# Autodesk Inventor assembly: Harmonic Drive - My Assembly
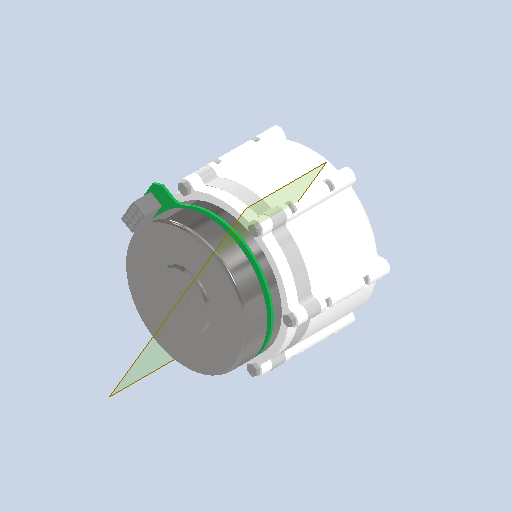
[picture p0: Inventor's stored thumbnail of the model, 512x512]
Saved by Autodesk Inventor 2023.2 (Build 272271000, 271)
## iProperties
Created: 2023-01-17
Part Number: Harmonic Drive - My Assembly
Document SubType Name: Assembly
Designer: Letícia
Author: Letícia
## Documents named in this file (27)
- C:\Users\User\Desktop\IC - Prof. Rafael\CADs\Redução Harmônica\HowToMechatronics\Harmonic Drive - PROJETO\Harmonic Drive - My Assembly.iam
- C:\Users\User\Desktop\IC - Prof. Rafael\CADs\Redução Harmônica\HowToMechatronics\Harmonic Drive - PROJETO\Housing.ipt
- C:\Users\User\Desktop\IC - Prof. Rafael\CADs\Redução Harmônica\HowToMechatronics\Harmonic Drive - PROJETO\4668K269.ipt
- C:\Users\User\Desktop\IC - Prof. Rafael\CADs\Redução Harmônica\HowToMechatronics\Harmonic Drive - PROJETO\BearingSpacer.ipt
- C:\Users\User\Desktop\IC - Prof. Rafael\CADs\Redução Harmônica\HowToMechatronics\Harmonic Drive - PROJETO\BearingSpacer2.ipt
- C:\Users\User\Desktop\IC - Prof. Rafael\CADs\Redução Harmônica\HowToMechatronics\Harmonic Drive - PROJETO\Spline output.ipt
- C:\Users\User\Desktop\IC - Prof. Rafael\CADs\Redução Harmônica\HowToMechatronics\Harmonic Drive - PROJETO\92010A230.ipt
- C:\Users\User\Desktop\IC - Prof. Rafael\CADs\Redução Harmônica\HowToMechatronics\Harmonic Drive - PROJETO\93475A230.ipt
- C:\Users\User\Desktop\IC - Prof. Rafael\CADs\Redução Harmônica\HowToMechatronics\Harmonic Drive - PROJETO\90576A103.ipt
- C:\Users\User\Desktop\IC - Prof. Rafael\CADs\Redução Harmônica\HowToMechatronics\Harmonic Drive - PROJETO\Output shaft.ipt
- C:\Users\User\Desktop\IC - Prof. Rafael\CADs\Redução Harmônica\HowToMechatronics\Harmonic Drive - PROJETO\91415A020.ipt
- C:\Users\User\Desktop\IC - Prof. Rafael\CADs\Redução Harmônica\HowToMechatronics\Harmonic Drive - PROJETO\92010A242.ipt
- C:\Users\User\Desktop\IC - Prof. Rafael\CADs\Redução Harmônica\HowToMechatronics\Harmonic Drive - PROJETO\Output.ipt
- C:\Users\User\Desktop\IC - Prof. Rafael\CADs\Redução Harmônica\HowToMechatronics\Harmonic Drive - PROJETO\91280A132.ipt
- C:\Users\User\Desktop\IC - Prof. Rafael\CADs\Redução Harmônica\HowToMechatronics\Harmonic Drive - PROJETO\Flex Spline.ipt
- C:\Users\User\Desktop\IC - Prof. Rafael\CADs\Redução Harmônica\HowToMechatronics\Harmonic Drive - PROJETO\Circular Spline.ipt
- C:\Users\User\Desktop\IC - Prof. Rafael\CADs\Redução Harmônica\HowToMechatronics\Harmonic Drive - PROJETO\Wave Generator p1.ipt
- C:\Users\User\Desktop\IC - Prof. Rafael\CADs\Redução Harmônica\HowToMechatronics\Harmonic Drive - PROJETO\Wave Generator p2.ipt
- C:\Users\User\Desktop\IC - Prof. Rafael\CADs\Redução Harmônica\HowToMechatronics\Harmonic Drive - PROJETO\4668K117.ipt
- C:\Users\User\Desktop\IC - Prof. Rafael\CADs\Redução Harmônica\HowToMechatronics\Harmonic Drive - PROJETO\92010A126.ipt
- C:\Users\User\Desktop\IC - Prof. Rafael\CADs\Redução Harmônica\HowToMechatronics\Harmonic Drive - PROJETO\90576A102.ipt
- C:\Users\User\Desktop\IC - Prof. Rafael\CADs\Redução Harmônica\HowToMechatronics\Harmonic Drive - PROJETO\Motor mount - Lid.ipt
- C:\Users\User\Desktop\IC - Prof. Rafael\CADs\Redução Harmônica\HowToMechatronics\Harmonic Drive - PROJETO\93695A120.ipt
- C:\Users\User\Desktop\IC - Prof. Rafael\CADs\Redução Harmônica\HowToMechatronics\Harmonic Drive - PROJETO\92605A102.ipt
- C:\Users\User\Desktop\IC - Prof. Rafael\Bancada\Motor Maxon323772_EC90fl_90W_A.ipt
- C:\Users\User\Documents\Inventor\Content Center Files\R2023\pt-BR\ANSI B18.6.5M(07)\ANSI B18.6.5M - 4.8x1.6 x 10(14).ipt
- C:\Users\User\Desktop\IC - Prof. Rafael\CADs\Redução Harmônica\HowToMechatronics\Harmonic Drive - PROJETO\91280A148.ipt
## Components (128 placed, 26 different names)
1. Housing:1 — Coincidente:1, Coincidente:2, Coincidente:4, Coincidente:8, Coincidente:11, Coincidente:12, Coincidente:13, Coincidente:14, Coincidente:41, Coincidente:42, Coincidente:43, Coincidente:44, Coincidente:45, Coincidente:143, Coincidente:144
2. 4668K269:1 — Coincidente:1, Coincidente:2, Coincidente:3, Coincidente:5, Coincidente:6, Coincidente:10
3. BearingSpacer:1 — Coincidente:3, Coincidente:4, Coincidente:7
4. BearingSpacer2:1 — Coincidente:5, Coincidente:6
5. Spline output:1 — Coincidente:9, Coincidente:10, Coincidente:18, Coincidente:19, Coincidente:20, Coincidente:21, Coincidente:22, Coincidente:23, Coincidente:32, Coincidente:34, Coincidente:35, Coincidente:36
6. Output shaft:1 — Coincidente:18, Coincidente:19, Coincidente:20, Coincidente:21, Coincidente:22, Coincidente:23, Coincidente:24, Coincidente:25, Coincidente:26, Coincidente:27, Coincidente:28, Coincidente:29
7. Output:1 — Coincidente:27, Coincidente:28, Coincidente:29, Coincidente:30, Coincidente:31
8. Flex Spline:1 — Coincidente:36, Coincidente:37, Coincidente:38, Coincidente:39
9. Circular Spline:1 — Coincidente:41, Coincidente:42, Coincidente:43, Coincidente:136, Coincidente:139, Coincidente:140, Coincidente:141
10. Wave Generator p1:1 — Coincidente:46, Coincidente:47, Coincidente:48, Coincidente:49, Coincidente:50, Coincidente:51, Coincidente:52, Coincidente:53, Coincidente:54, Coincidente:55, Coincidente:56, Coincidente:57, Coincidente:58, Coincidente:59, Coincidente:60, Coincidente:61, Coincidente:62, Coincidente:63, Coincidente:64, Coincidente:65, Coincidente:66, Coincidente:67, Coincidente:68, Coincidente:69, Coincidente:70, Coincidente:71, Coincidente:72, Coincidente:73, Coincidente:74, Coincidente:75, Coincidente:76, Coincidente:77, Coincidente:78, Coincidente:79, Coincidente:80, Coincidente:81, Coincidente:82, Coincidente:83, Coincidente:84, Coincidente:85, Coincidente:86, Coincidente:87, Coincidente:88, Coincidente:109, Coincidente:110, Coincidente:111, Coincidente:112, Coincidente:114, Coincidente:116, Coincidente:117, Coincidente:118, Coincidente:119, Coincidente:120, Coincidente:121, Coincidente:122, Coincidente:134, Coincidente:135
11. Wave Generator p2:1 — Coincidente:66, Coincidente:67, Coincidente:68, Coincidente:90, Coincidente:92, Coincidente:94, Coincidente:96, Coincidente:98, Coincidente:100, Coincidente:102, Coincidente:104, Coincidente:106, Coincidente:108, Coincidente:126, Coincidente:127, Coincidente:138
12. 4668K117:8 — Coincidente:46, Coincidente:47
13. 4668K117:9 — Coincidente:48, Coincidente:49
14. 4668K117:10 — Coincidente:64, Coincidente:65
15. 4668K117:11 — Coincidente:62, Coincidente:63
16. 4668K117:12 — Coincidente:60, Coincidente:61
17. 4668K117:13 — Coincidente:58, Coincidente:59
18. 4668K117:14 — Coincidente:56, Coincidente:57
19. 4668K117:15 — Coincidente:54, Coincidente:55
20. 4668K117:16 — Coincidente:52, Coincidente:53
21. 4668K117:17 — Coincidente:50, Coincidente:51
22. 92010A126:1 — Coincidente:75, Coincidente:76, Coincidente:107
23. 92010A126:2 — Coincidente:73, Coincidente:74, Coincidente:97
24. 92010A126:3 — Coincidente:71, Coincidente:72, Coincidente:95
25. 92010A126:4 — Coincidente:69, Coincidente:70, Coincidente:93
26. 92010A126:5 — Coincidente:87, Coincidente:88, Coincidente:89
27. 92010A126:6 — Coincidente:85, Coincidente:86, Coincidente:91
28. 92010A126:7 — Coincidente:83, Coincidente:84, Coincidente:105
29. 92010A126:8 — Coincidente:81, Coincidente:82, Coincidente:103
30. 92010A126:9 — Coincidente:79, Coincidente:80, Coincidente:101
31. 92010A126:10 — Coincidente:77, Coincidente:78, Coincidente:99
32. 90576A102:1 — Coincidente:89, Coincidente:90
33. 90576A102:2 — Coincidente:91, Coincidente:92
34. 90576A102:3 — Coincidente:105, Coincidente:106
35. 90576A102:4 — Coincidente:103, Coincidente:104
36. 90576A102:5 — Coincidente:101, Coincidente:102
37. 90576A102:6 — Coincidente:99, Coincidente:100
38. 90576A102:7 — Coincidente:107, Coincidente:108
39. 90576A102:8 — Coincidente:97, Coincidente:98
40. 90576A102:9 — Coincidente:95, Coincidente:96
41. 90576A102:10 — Coincidente:93, Coincidente:94
42. Motor mount - Lid:1 — Coincidente:128, Coincidente:129, Coincidente:130, Coincidente:131, Coincidente:132, Coincidente:133, Coincidente:134, Coincidente:136, Coincidente:139, Coincidente:140, Coincidente:142
43. 93695A120:1 — Coincidente:109, Coincidente:110, Coincidente:113
44. 93695A120:2 — Coincidente:111, Coincidente:112, Coincidente:115
45. 92605A102:1 — Coincidente:113, Coincidente:114
46. 92605A102:2 — Coincidente:115, Coincidente:116
47. 92010A126:11 — Coincidente:119, Coincidente:120, Coincidente:123
48. 92010A126:12 — Coincidente:121, Coincidente:122, Coincidente:137
49. 92010A126:13 — Coincidente:117, Coincidente:118, Coincidente:125
50. 90576A102:11 — Coincidente:123, Coincidente:127
51. 90576A102:13 — Coincidente:125, Coincidente:126
52. Motor Maxon323772_EC90fl_90W_A:1 — Coincidente:128, Coincidente:129, Coincidente:130, Coincidente:135, Flush:1
53. Parafuso Phillips para chapa de cabeça escareada reta - Tipo BT - Tipo IA - Métrica 4.8x1.6 x 10:1 — Coincidente:131
54. Parafuso Phillips para chapa de cabeça escareada reta - Tipo BT - Tipo IA - Métrica 4.8x1.6 x 10:2 — Coincidente:132
55. Parafuso Phillips para chapa de cabeça escareada reta - Tipo BT - Tipo IA - Métrica 4.8x1.6 x 10:3 — Coincidente:133
56. 90576A102:14 — Coincidente:137, Coincidente:138
57. 92010A230:1 — Coincidente:11, Coincidente:12, Coincidente:13, Coincidente:15, Coincidente:17
58. 4668K269:2 — Coincidente:7, Coincidente:8, Coincidente:9
59. 92010A230:7
60. 4668K269:3
61. 92010A230:8
62. 4668K269:4
63. 92010A230:9
64. 4668K269:5
65. 92010A230:10
66. 4668K269:6
67. 92010A230:11
68. 4668K269:7
69. 93475A230:1 — Coincidente:14, Coincidente:15, Coincidente:16
70. 93475A230:2
71. 93475A230:3
72. 93475A230:4
73. 93475A230:5
74. 93475A230:6
75. 90576A103:1 — Coincidente:16, Coincidente:17
76. 90576A103:2
77. 90576A103:3
78. 90576A103:4
79. 90576A103:5
80. 90576A103:6
81. 91415A020:1 — Coincidente:24, Coincidente:25, Coincidente:26
82. 91415A020:2
83. 91415A020:3
84. 91415A020:4
85. 92010A242:1 — Coincidente:30, Coincidente:31
86. 92010A242:2 — Coincidente:33
87. 92010A242:3
88. 92010A242:4
89. 90576A103:7 — Coincidente:32, Coincidente:33
90. 90576A103:8
91. 90576A103:9
92. 90576A103:10
93. 91280A132:1 — Coincidente:34, Coincidente:35
94. 91280A132:2
95. 91280A132:3
96. 91280A132:4 — Coincidente:40
97. 91280A132:5 — Coincidente:38
98. 91280A132:6 — Coincidente:37
99. 90576A103:11 — Coincidente:39, Coincidente:40
100. 90576A103:12
101. 90576A103:13
102. 90576A103:14
103. 90576A103:15
104. 90576A103:16
105. 91415A020:5 — Coincidente:44, Coincidente:45
106. 91415A020:6
107. 91415A020:7
108. 91415A020:8
109. 91415A020:9
110. 91415A020:10
111. 91280A148:2 — Coincidente:141, Coincidente:142
112. 91280A148:3
113. 91280A148:4
114. 91280A148:5
115. 91280A148:6
116. 91280A148:7
117. 91415A020:11 — Coincidente:143, Coincidente:144
118. 91415A020:12
119. 91415A020:13
120. 91415A020:14
121. 91415A020:15
122. 91415A020:16
123. 91415A020:17
124. 91415A020:18
125. 91415A020:19
126. 91415A020:20
127. 91415A020:21
128. 91415A020:22
## Component patterns: (6 elements, first: 92010A230:1 + 4668K269:2), (6 elements, first: 93475A230:1), (6 elements, first: 90576A103:1), (4 elements, first: 91415A020:1), (4 elements, first: 92010A242:1), (4 elements, first: 90576A103:7), (6 elements, first: 91280A132:1), (6 elements, first: 90576A103:11), (6 elements, first: 91415A020:5), (6 elements, first: 91280A148:2), (6 elements), (2 elements, first: 91415A020:11), Componente de padrão 11:2 (2 elements), Componente de padrão 11:3 (2 elements), Componente de padrão 11:4 (2 elements), Componente de padrão 11:5 (2 elements), Componente de padrão 11:6 (2 elements)
## Relationships (144: Mate 143, Flush 1)
- Coincidente:1 [Mate]: Housing:1 ↔ 4668K269:1
- Coincidente:2 [Mate]: Housing:1 ↔ 4668K269:1
- Coincidente:3 [Mate]: 4668K269:1 ↔ BearingSpacer:1
- Coincidente:4 [Mate]: Housing:1 ↔ BearingSpacer:1
- Coincidente:5 [Mate]: 4668K269:1 ↔ BearingSpacer2:1
- Coincidente:6 [Mate]: 4668K269:1 ↔ BearingSpacer2:1
- Coincidente:7 [Mate]: BearingSpacer:1 ↔ 4668K269:2
- Coincidente:8 [Mate]: Housing:1 ↔ 4668K269:2
- Coincidente:9 [Mate]: Spline output:1 ↔ 4668K269:2
- Coincidente:10 [Mate]: 4668K269:1 ↔ Spline output:1
- Coincidente:11 [Mate]: Housing:1 ↔ 92010A230:1
- Coincidente:12 [Mate]: Housing:1 ↔ 92010A230:1
- Coincidente:13 [Mate]: Housing:1 ↔ 92010A230:1
- Coincidente:14 [Mate]: Housing:1 ↔ 93475A230:1
- Coincidente:15 [Mate]: 92010A230:1 ↔ 93475A230:1
- Coincidente:16 [Mate]: 93475A230:1 ↔ 90576A103:1
- Coincidente:17 [Mate]: 92010A230:1 ↔ 90576A103:1
- Coincidente:18 [Mate]: Spline output:1 ↔ Output shaft:1
- Coincidente:19 [Mate]: Spline output:1 ↔ Output shaft:1
- Coincidente:20 [Mate]: Spline output:1 ↔ Output shaft:1
- Coincidente:21 [Mate]: Spline output:1 ↔ Output shaft:1
- Coincidente:22 [Mate]: Spline output:1 ↔ Output shaft:1
- Coincidente:23 [Mate]: Spline output:1 ↔ Output shaft:1
- Coincidente:24 [Mate]: Output shaft:1 ↔ 91415A020:1
- Coincidente:25 [Mate]: Output shaft:1 ↔ 91415A020:1
- Coincidente:26 [Mate]: Output shaft:1 ↔ 91415A020:1
- Coincidente:27 [Mate]: Output shaft:1 ↔ Output:1
- Coincidente:28 [Mate]: Output shaft:1 ↔ Output:1
- Coincidente:29 [Mate]: Output shaft:1 ↔ Output:1
- Coincidente:30 [Mate]: Output:1 ↔ 92010A242:1
- Coincidente:31 [Mate]: Output:1 ↔ 92010A242:1
- Coincidente:32 [Mate]: Spline output:1 ↔ 90576A103:7
- Coincidente:33 [Mate]: 92010A242:2 ↔ 90576A103:7
- Coincidente:34 [Mate]: Spline output:1 ↔ 91280A132:1
- Coincidente:35 [Mate]: Spline output:1 ↔ 91280A132:1
- Coincidente:36 [Mate]: Spline output:1 ↔ Flex Spline:1
- Coincidente:37 [Mate]: Flex Spline:1 ↔ 91280A132:6
- Coincidente:38 [Mate]: Flex Spline:1 ↔ 91280A132:5
- Coincidente:39 [Mate]: Flex Spline:1 ↔ 90576A103:11
- Coincidente:40 [Mate]: 91280A132:4 ↔ 90576A103:11
- Coincidente:41 [Mate]: Housing:1 ↔ Circular Spline:1
- Coincidente:42 [Mate]: Housing:1 ↔ Circular Spline:1
- Coincidente:43 [Mate]: Housing:1 ↔ Circular Spline:1
- Coincidente:44 [Mate]: Housing:1 ↔ 91415A020:5
- Coincidente:45 [Mate]: Housing:1 ↔ 91415A020:5
- Coincidente:46 [Mate]: Wave Generator p1:1 ↔ 4668K117:8
- Coincidente:47 [Mate]: Wave Generator p1:1 ↔ 4668K117:8
- Coincidente:48 [Mate]: Wave Generator p1:1 ↔ 4668K117:9
- Coincidente:49 [Mate]: Wave Generator p1:1 ↔ 4668K117:9
- Coincidente:50 [Mate]: Wave Generator p1:1 ↔ 4668K117:17
- Coincidente:51 [Mate]: Wave Generator p1:1 ↔ 4668K117:17
- Coincidente:52 [Mate]: Wave Generator p1:1 ↔ 4668K117:16
- Coincidente:53 [Mate]: Wave Generator p1:1 ↔ 4668K117:16
- Coincidente:54 [Mate]: Wave Generator p1:1 ↔ 4668K117:15
- Coincidente:55 [Mate]: Wave Generator p1:1 ↔ 4668K117:15
- Coincidente:56 [Mate]: Wave Generator p1:1 ↔ 4668K117:14
- Coincidente:57 [Mate]: Wave Generator p1:1 ↔ 4668K117:14
- Coincidente:58 [Mate]: Wave Generator p1:1 ↔ 4668K117:13
- Coincidente:59 [Mate]: Wave Generator p1:1 ↔ 4668K117:13
- Coincidente:60 [Mate]: Wave Generator p1:1 ↔ 4668K117:12
- Coincidente:61 [Mate]: Wave Generator p1:1 ↔ 4668K117:12
- Coincidente:62 [Mate]: Wave Generator p1:1 ↔ 4668K117:11
- Coincidente:63 [Mate]: Wave Generator p1:1 ↔ 4668K117:11
- Coincidente:64 [Mate]: Wave Generator p1:1 ↔ 4668K117:10
- Coincidente:65 [Mate]: Wave Generator p1:1 ↔ 4668K117:10
- Coincidente:66 [Mate]: Wave Generator p1:1 ↔ Wave Generator p2:1
- Coincidente:67 [Mate]: Wave Generator p1:1 ↔ Wave Generator p2:1
- Coincidente:68 [Mate]: Wave Generator p1:1 ↔ Wave Generator p2:1
- Coincidente:69 [Mate]: Wave Generator p1:1 ↔ 92010A126:4
- Coincidente:70 [Mate]: Wave Generator p1:1 ↔ 92010A126:4
- Coincidente:71 [Mate]: Wave Generator p1:1 ↔ 92010A126:3
- Coincidente:72 [Mate]: Wave Generator p1:1 ↔ 92010A126:3
- Coincidente:73 [Mate]: Wave Generator p1:1 ↔ 92010A126:2
- Coincidente:74 [Mate]: Wave Generator p1:1 ↔ 92010A126:2
- Coincidente:75 [Mate]: Wave Generator p1:1 ↔ 92010A126:1
- Coincidente:76 [Mate]: Wave Generator p1:1 ↔ 92010A126:1
- Coincidente:77 [Mate]: Wave Generator p1:1 ↔ 92010A126:10
- Coincidente:78 [Mate]: Wave Generator p1:1 ↔ 92010A126:10
- Coincidente:79 [Mate]: Wave Generator p1:1 ↔ 92010A126:9
- Coincidente:80 [Mate]: Wave Generator p1:1 ↔ 92010A126:9
- Coincidente:81 [Mate]: Wave Generator p1:1 ↔ 92010A126:8
- Coincidente:82 [Mate]: Wave Generator p1:1 ↔ 92010A126:8
- Coincidente:83 [Mate]: Wave Generator p1:1 ↔ 92010A126:7
- Coincidente:84 [Mate]: Wave Generator p1:1 ↔ 92010A126:7
- Coincidente:85 [Mate]: Wave Generator p1:1 ↔ 92010A126:6
- Coincidente:86 [Mate]: Wave Generator p1:1 ↔ 92010A126:6
- Coincidente:87 [Mate]: Wave Generator p1:1 ↔ 92010A126:5
- Coincidente:88 [Mate]: Wave Generator p1:1 ↔ 92010A126:5
- Coincidente:89 [Mate]: 92010A126:5 ↔ 90576A102:1
- Coincidente:90 [Mate]: Wave Generator p2:1 ↔ 90576A102:1
- Coincidente:91 [Mate]: 92010A126:6 ↔ 90576A102:2
- Coincidente:92 [Mate]: Wave Generator p2:1 ↔ 90576A102:2
- Coincidente:93 [Mate]: 92010A126:4 ↔ 90576A102:10
- Coincidente:94 [Mate]: Wave Generator p2:1 ↔ 90576A102:10
- Coincidente:95 [Mate]: 92010A126:3 ↔ 90576A102:9
- Coincidente:96 [Mate]: Wave Generator p2:1 ↔ 90576A102:9
- Coincidente:97 [Mate]: 92010A126:2 ↔ 90576A102:8
- Coincidente:98 [Mate]: Wave Generator p2:1 ↔ 90576A102:8
- Coincidente:99 [Mate]: 92010A126:10 ↔ 90576A102:6
- Coincidente:100 [Mate]: Wave Generator p2:1 ↔ 90576A102:6
- Coincidente:101 [Mate]: 92010A126:9 ↔ 90576A102:5
- Coincidente:102 [Mate]: Wave Generator p2:1 ↔ 90576A102:5
- Coincidente:103 [Mate]: 92010A126:8 ↔ 90576A102:4
- Coincidente:104 [Mate]: Wave Generator p2:1 ↔ 90576A102:4
- Coincidente:105 [Mate]: 92010A126:7 ↔ 90576A102:3
- Coincidente:106 [Mate]: Wave Generator p2:1 ↔ 90576A102:3
- Coincidente:107 [Mate]: 92010A126:1 ↔ 90576A102:7
- Coincidente:108 [Mate]: Wave Generator p2:1 ↔ 90576A102:7
- Coincidente:109 [Mate]: Wave Generator p1:1 ↔ 93695A120:1
- Coincidente:110 [Mate]: Wave Generator p1:1 ↔ 93695A120:1
- Coincidente:111 [Mate]: Wave Generator p1:1 ↔ 93695A120:2
- Coincidente:112 [Mate]: Wave Generator p1:1 ↔ 93695A120:2
- Coincidente:113 [Mate]: 93695A120:1 ↔ 92605A102:1
- Coincidente:114 [Mate] (4 mm): Wave Generator p1:1 ↔ 92605A102:1
- Coincidente:115 [Mate]: 93695A120:2 ↔ 92605A102:2
- Coincidente:116 [Mate] (4 mm): Wave Generator p1:1 ↔ 92605A102:2
- Coincidente:117 [Mate]: Wave Generator p1:1 ↔ 92010A126:13
- Coincidente:118 [Mate]: Wave Generator p1:1 ↔ 92010A126:13
- Coincidente:119 [Mate]: Wave Generator p1:1 ↔ 92010A126:11
- Coincidente:120 [Mate]: Wave Generator p1:1 ↔ 92010A126:11
- Coincidente:121 [Mate]: Wave Generator p1:1 ↔ 92010A126:12
- Coincidente:122 [Mate]: Wave Generator p1:1 ↔ 92010A126:12
- Coincidente:123 [Mate]: 92010A126:11 ↔ 90576A102:11
- Coincidente:125 [Mate]: 92010A126:13 ↔ 90576A102:13
- Coincidente:126 [Mate]: Wave Generator p2:1 ↔ 90576A102:13
- Coincidente:127 [Mate]: Wave Generator p2:1 ↔ 90576A102:11
- Coincidente:128 [Mate]: Motor mount - Lid:1 ↔ Motor Maxon323772_EC90fl_90W_A:1
- Coincidente:129 [Mate]: Motor mount - Lid:1 ↔ Motor Maxon323772_EC90fl_90W_A:1
- Coincidente:130 [Mate]: Motor mount - Lid:1 ↔ Motor Maxon323772_EC90fl_90W_A:1
- Coincidente:131 [Mate]: Motor mount - Lid:1 ↔ Parafuso Phillips para chapa de cabeça escareada reta - Tipo BT - Tipo IA - Métrica 4.8x1.6 x 10:1
- Coincidente:132 [Mate]: Motor mount - Lid:1 ↔ Parafuso Phillips para chapa de cabeça escareada reta - Tipo BT - Tipo IA - Métrica 4.8x1.6 x 10:2
- Coincidente:133 [Mate]: Motor mount - Lid:1 ↔ Parafuso Phillips para chapa de cabeça escareada reta - Tipo BT - Tipo IA - Métrica 4.8x1.6 x 10:3
- Coincidente:134 [Mate]: Wave Generator p1:1 ↔ Motor mount - Lid:1
- Coincidente:135 [Mate]: Wave Generator p1:1 ↔ Motor Maxon323772_EC90fl_90W_A:1
- Coincidente:136 [Mate]: Circular Spline:1 ↔ Motor mount - Lid:1
- Coincidente:137 [Mate]: 92010A126:12 ↔ 90576A102:14
- Coincidente:138 [Mate]: Wave Generator p2:1 ↔ 90576A102:14
- Coincidente:139 [Mate]: Circular Spline:1 ↔ Motor mount - Lid:1
- Coincidente:140 [Mate]: Circular Spline:1 ↔ Motor mount - Lid:1
- Coincidente:141 [Mate]: Circular Spline:1 ↔ 91280A148:2
- Coincidente:142 [Mate]: Motor mount - Lid:1 ↔ 91280A148:2
- Coincidente:143 [Mate]: Housing:1 ↔ 91415A020:11
- Coincidente:144 [Mate]: Housing:1 ↔ 91415A020:11
- Flush:1 (-57 mm): Motor Maxon323772_EC90fl_90W_A:1
